# Autodesk Inventor assembly: Ensamblaje1
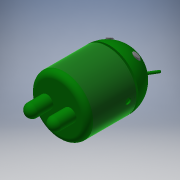
[picture p0: Inventor's stored thumbnail of the model, 180x180]
Saved by Autodesk Inventor 2016 (Build 200138000, 138)
## iProperties
Created: 2016-02-20
Part Number: Ensamblaje1
Material: Genérico
Document SubType Name: Assembly
Designer: Usuario1
Author: Usuario1
## Documents named in this file (7)
- C:\Users\Usuario1\Desktop\sol\3d\android\Ensamblaje1.iam
- C:\Users\Usuario1\Desktop\sol\3d\android\pie.ipt
- C:\Users\Usuario1\Desktop\sol\3d\android\cuerpo.ipt
- C:\Users\Usuario1\Desktop\sol\3d\android\cuello.ipt
- C:\Users\Usuario1\Desktop\sol\3d\android\enlacecuello.ipt
- C:\Users\Usuario1\Desktop\sol\3d\android\cabeza.ipt
- C:\Users\Usuario1\Desktop\sol\3d\android\ojos.ipt
## Components (7 placed, 6 different names)
1. pie:1 — Coincidencia:1
2. pie:2 — Coincidencia:2
3. cuerpo:1 — Coincidencia:1, Coincidencia:2, Coincidencia:3
4. cuello:1 — Coincidencia:3, Coincidencia:4
5. enlacecuello:1 — Coincidencia:4, Rígido:1
6. cabeza:1 — Coincidencia:5, Rígido:1
7. ojos:1 — Coincidencia:5
## Relationships (6: Mate 5, WeldJoint 1)
- Coincidencia:1 [Mate]: pie:1 ↔ cuerpo:1
- Coincidencia:2 [Mate]: pie:2 ↔ cuerpo:1
- Coincidencia:3 [Mate]: cuerpo:1 ↔ cuello:1
- Coincidencia:4 [Mate]: cuello:1 ↔ enlacecuello:1
- Coincidencia:5 [Mate]: cabeza:1 ↔ ojos:1
- Rígido:1 [WeldJoint]: enlacecuello:1 ↔ cabeza:1
